# Autodesk Inventor assembly: untitled.brd
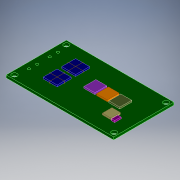
[picture p0: Inventor's stored thumbnail of the model, 180x180]
Saved by Autodesk Inventor 2022 (Build 260153000, 153)
## iProperties
Created: 2023-03-06
Part Number: untitled.brd
Document SubType Name: Assembly
Designer: Иван Петров
Author: Иван Петров
## Documents named in this file (10)
- C:\Users\Ivan Petrov\Documents\GitHub\OmniBot\electronic\3V_power_board\3d model\untitled.brd.iam
- C:\Users\Ivan Petrov\Documents\GitHub\OmniBot\electronic\3V_power_board\3d model\untitled.brdКонтур.ipt
- C:\Users\Ivan Petrov\Documents\GitHub\OmniBot\electronic\3V_power_board\3d model\153CLV-0810, 153CLV-0810_1.ipt
- C:\Users\Ivan Petrov\Documents\GitHub\OmniBot\electronic\3V_power_board\3d model\SCREWTERMINAL-5MM-2, J1_SCREWTERMINAL-5MM-2_4.ipt
- C:\Users\Ivan Petrov\Documents\GitHub\OmniBot\electronic\3V_power_board\3d model\SCREWTERMINAL-5MM-2, J2_SCREWTERMINAL-5MM-2_6.ipt
- C:\Users\Ivan Petrov\Documents\GitHub\OmniBot\electronic\3V_power_board\3d model\LED5MM, LED5MM_8.ipt
- C:\Users\Ivan Petrov\Documents\GitHub\OmniBot\electronic\3V_power_board\3d model\R0805, R0805_10.ipt
- C:\Users\Ivan Petrov\Documents\GitHub\OmniBot\electronic\3V_power_board\3d model\SOT223, U1_SOT223_12.ipt
- C:\Users\Ivan Petrov\Documents\GitHub\OmniBot\electronic\3V_power_board\3d model\SOT223, U2_SOT223_14.ipt
- C:\Users\Ivan Petrov\Documents\GitHub\OmniBot\electronic\3V_power_board\3d model\SOT223, U3_SOT223_16.ipt
## Components (10 placed, 10 different names)
1. untitled.brdКонтур:1
2. C9_2 — Совмещение:5, Угол:3, Совмещение:6, Угол:4
3. C10_3 — Совмещение:1, Угол:1, Совмещение:2, Угол:2
4. J1_5
5. J2_7
6. LED2_9
7. R6_11
8. U1_13
9. U2_15
10. U3_17
## Relationships (12: Mate 8, Angle 4)
- Совмещение:1 [Mate]: C10_3
- Угол:1 [Angle] (0 deg): C10_3
- Совмещение:2 [Mate]: C10_3
- Угол:2 [Angle] (0 deg): C10_3
- Совмещение:3 [Mate]
- Совмещение:4 [Mate]
- Совмещение:5 [Mate]: C9_2
- Угол:3 [Angle] (0 deg): C9_2
- Совмещение:6 [Mate]: C9_2
- Угол:4 [Angle] (0 deg): C9_2
- Совмещение:7 [Mate]
- Совмещение:8 [Mate]
